# Autodesk Inventor assembly: 6 in Traction Tire
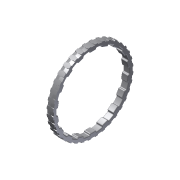
[picture p0: Inventor's stored thumbnail of the model, 180x180]
Saved by Autodesk Inventor 2013 (Build 170138000, 138)
## iProperties
Created: 2013-12-23
Part Number: 6 in Traction Tire
Document SubType Name: Assembly
Designer: Nemo
Author: Nemo
## Documents named in this file (3)
- H:\Nemo\Documents\Robotics\COTS Parts\Wheels\VexPro Traction Wheels\Components\6 in Traction Tire.iam
- H:\Nemo\Documents\Robotics\COTS Parts\Wheels\VexPro Traction Wheels\Components\6 in Traction Tire insert.ipt
- H:\Nemo\Documents\Robotics\COTS Parts\Wheels\VexPro Traction Wheels\Components\6 in Traction Tire Tread.ipt
## Components (2 placed, 2 different names)
1. 6 in Traction Tire insert:1 — Mate:1, Flush:1, Angle:1, Mate:3
2. 6 in Traction Tire Tread:1 — Mate:2, Mate:3, Flush:2
## Relationships (6: Mate 3, Flush 2, Angle 1)
- Mate:1: 6 in Traction Tire insert:1
- Flush:1: 6 in Traction Tire insert:1
- Angle:1 (10 deg): 6 in Traction Tire insert:1
- Mate:2: 6 in Traction Tire Tread:1
- Mate:3: 6 in Traction Tire insert:1 ↔ 6 in Traction Tire Tread:1
- Flush:2: 6 in Traction Tire Tread:1
